# Autodesk Inventor assembly: BAO Sign
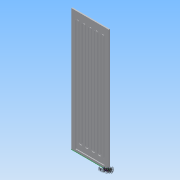
[picture p0: Inventor's stored thumbnail of the model, 180x180]
Saved by Autodesk Inventor 2013 (Build 170138000, 138)
## iProperties
Created: 2018-07-18
Part Number: BAO Sign
Document SubType Name: Assembly
Designer: Jeff Vyduna
Author: Jeff Vyduna
## Documents named in this file (3)
- \\vmware-host\Shared Folders\Desktop\Hot fresh bao sign\CAD\NWOW\BAO Sign.iam
- \\vmware-host\Shared Folders\Desktop\Hot fresh bao sign\CAD\NWOW\Sign ply back, v3 separate parts.ipt
- \\vmware-host\Shared Folders\Desktop\Hot fresh bao sign\CAD\NWOW\Sideborder.ipt
## Components (1 placed, 1 different names)
1. Ply back
## Named parameters: signW = 609.6 mm, borderLap = 12.7 mm, borderW = 38.1 mm, borderH = 25.4 mm, velcroH = 2.54 mm, panelH = 5.1308 mm, panelHClear = 0.79375 mm, signH = 1981.2 mm
